# Autodesk Inventor assembly: RS775+gennsoku
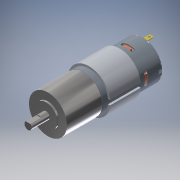
[picture p0: Inventor's stored thumbnail of the model, 180x180]
Saved by Autodesk Inventor 2019 (Build 230136000, 136)
## iProperties
Created: 2022-02-27
Part Number: RS775+gennsoku
Material: 一般
Document SubType Name: Assembly
Designer: yuta
Author: yuta
## Documents named in this file (3)
- C:\Users\yuta\Documents\NHK\RS775+gennsoku.iam
- C:\Users\yuta\Documents\NHK\RS775_CAD_IAM\モーター RS775-8513DF.iam
- C:\Users\yuta\Documents\NHK\nhk_gensoku.ipt
## Components (2 placed, 2 different names)
1. モーター RS775-8513DF:1 [sub-assembly] — メイト:1, メイト:2
2. nhk_gensoku:1 — メイト:1, メイト:2
## Relationships (2: Mate 2)
- メイト:1 [Mate]: モーター RS775-8513DF:1 ↔ nhk_gensoku:1
- メイト:2 [Mate]: モーター RS775-8513DF:1 ↔ nhk_gensoku:1
